# Autodesk Inventor assembly: Förderband
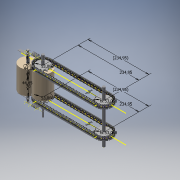
[picture p0: Inventor's stored thumbnail of the model, 180x180]
Saved by Autodesk Inventor 2018 (Build 220112000, 112)
## iProperties
Created: 2018-01-11
Part Number: Förderband
Material: Generisch
Document SubType Name: Assembly
Designer: Dominik
Author: Dominik
## Documents named in this file (6)
- C:\Users\Julian\Desktop\Schule\5AHME\Diplomarbeit\Git\fuettr_prototype\Mechanical\Inventorskizzen\Förderband.iam
- C:\Users\Julian\Desktop\Schule\5AHME\Diplomarbeit\Git\fuettr_prototype\Mechanical\Inventorskizzen\Kettenradzusammensetzung_links.iam
- C:\Users\Julian\Desktop\Schule\5AHME\Diplomarbeit\Git\fuettr_prototype\Mechanical\Inventorskizzen\Förderbandwelle_vorne.ipt
- C:\Users\Julian\Desktop\Schule\5AHME\Diplomarbeit\Git\fuettr_prototype\Mechanical\Inventorskizzen\Förderbandwelle_hinten.ipt
- C:\Users\Julian\Desktop\Schule\5AHME\Diplomarbeit\Git\fuettr_prototype\Mechanical\Inventorskizzen\Kunststoffrolle_antrieb.ipt
- C:\Users\Julian\Desktop\Schule\5AHME\Diplomarbeit\Git\fuettr_prototype\Mechanical\Inventorskizzen\Auspressrolle_befaesstigung.iam
## Components (6 placed, 5 different names)
1. Kettenradzusammensetzung_links:1 [sub-assembly] — Starr:2, Starr:5
2. Kettenradzusammensetzung_links:2 [sub-assembly] — Starr:1, Starr:4
3. Kunststoffrolle_antrieb:1 — Starr:3
4. Förderbandwelle_hinten:1 — Starr:4, Starr:5
5. Förderbandwelle_vorne:1 — Starr:1, Starr:2, Starr:3, Drehbar:1
6. Auspressrolle_befaesstigung:1 [sub-assembly] — Drehbar:1
## Relationships (6: WeldJoint 5, RevoluteJoint 1)
- Starr:1 [WeldJoint]: Kettenradzusammensetzung_links:2 ↔ Förderbandwelle_vorne:1
- Starr:2 [WeldJoint]: Kettenradzusammensetzung_links:1 ↔ Förderbandwelle_vorne:1
- Starr:3 [WeldJoint]: Kunststoffrolle_antrieb:1 ↔ Förderbandwelle_vorne:1
- Starr:4 [WeldJoint]: Kettenradzusammensetzung_links:2 ↔ Förderbandwelle_hinten:1
- Starr:5 [WeldJoint]: Kettenradzusammensetzung_links:1 ↔ Förderbandwelle_hinten:1
- Drehbar:1 [RevoluteJoint]: Förderbandwelle_vorne:1 ↔ Auspressrolle_befaesstigung:1
